# Autodesk Inventor assembly: Assembly_MicroscopeInABox_v0
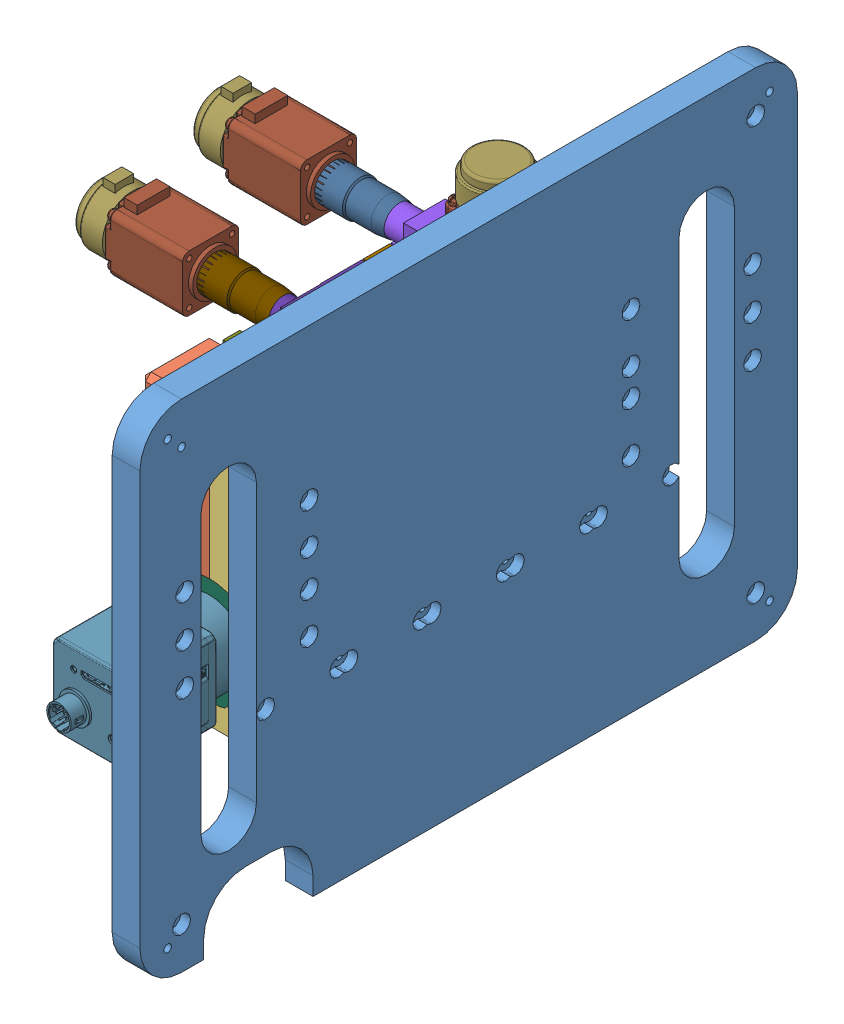
[picture p0: shaded view drawn from the shape stored in the file]
Saved by Autodesk Inventor 2024.1 (Build 281209000, 209)
## iProperties
Created: 2024-08-15
Part Number: Assembly_MicroscopeInABox_v0
Document SubType Name: Assembly
Designer: diederichbenedict
Author: diederichbenedict
## Documents named in this file (9)
- C:\Users\diederichbenedict\Dropbox\Dokumente\Promotion\PROJECTS\openUC2_SOOP\INVENTOR\Workspace\Assembly_MicroscopeInABox_v0.iam
- C:\Users\diederichbenedict\Dropbox\Dokumente\Promotion\PROJECTS\openUC2_SOOP\INVENTOR\Workspace\00_HIKCamera_MV-CE060-10UMUC\00_HIKCamera_MV-CE060-10UMUC.ipt
- C:\Users\diederichbenedict\Dropbox\Dokumente\Promotion\PROJECTS\openUC2_SOOP\INVENTOR\Workspace\00_10x_Objective_ViewSolutions_bm05073332.ipt
- C:\Users\diederichbenedict\Dropbox\Dokumente\Promotion\PROJECTS\openUC2_SOOP\INVENTOR\Workspace\00_Berrybase_CCTVLens_50mm.ipt
- C:\Users\diederichbenedict\Dropbox\Dokumente\Promotion\PROJECTS\openUC2_SOOP\INVENTOR\Workspace\Assembly_XYZ_Stage_Micrometer_ontop_lightsheet.iam
- C:\Users\diederichbenedict\Dropbox\Dokumente\Promotion\PROJECTS\openUC2_SOOP\INVENTOR\Workspace\MIAB_Case_v0.ipt
- C:\Users\diederichbenedict\Dropbox\Dokumente\Promotion\PROJECTS\openUC2_SOOP\INVENTOR\Workspace\MIAB_Case_Opticscube_RMS_1.ipt
- C:\Users\diederichbenedict\Dropbox\Dokumente\Promotion\PROJECTS\openUC2_SOOP\INVENTOR\Workspace\MIAB_Case_v0_MIR.ipt
- C:\Users\diederichbenedict\Dropbox\Dokumente\Promotion\PROJECTS\openUC2_SOOP\INVENTOR\Workspace\60_Planktoscope_MicroscopeHolderXYZ_Bottom_v0.ipt
## Components (8 placed, 8 different names)
1. 00_HIKCamera_MV-CE060-10UMUC:1 — Einfügen:2, Winkel:1
2. 00_10x_Objective_ViewSolutions_bm05073332:1 — Passend:1, Fluchtend:1, Einfügen:1, Passend:2
3. 00_Berrybase_CCTVLens_50mm:1 — Einfügen:1, Einfügen:2, Passend:3
4. Assembly_XYZ_Stage_Micrometer_ontop_lightsheet:1 [sub-assembly] — Passend:2, Winkel:2, Passend:3
5. MIAB_Case_v0:1 — Fluchtend:2, Fluchtend:3, Fluchtend:4, Fluchtend:5, Passend:6, Fluchtend:6, Fluchtend:7
6. MIAB_Case_Opticscube_RMS_1:1 — Fluchtend:4, Fluchtend:5
7. MIAB_Case_v0_MIR:1 — Passend:4, Passend:5
8. 60_Planktoscope_MicroscopeHolderXYZ_Bottom_v0:1 — Passend:6, Fluchtend:6, Fluchtend:7
## Relationships (17: Flush 7, Mate 6, Insert 2, Angle 2)
- Passend:1 [Mate]: 00_10x_Objective_ViewSolutions_bm05073332:1
- Fluchtend:1 [Flush]: 00_10x_Objective_ViewSolutions_bm05073332:1
- Einfügen:1 [Insert] (25 mm): 00_10x_Objective_ViewSolutions_bm05073332:1 ↔ 00_Berrybase_CCTVLens_50mm:1
- Einfügen:2 [Insert]: 00_HIKCamera_MV-CE060-10UMUC:1 ↔ 00_Berrybase_CCTVLens_50mm:1
- Winkel:1 [Angle] (0 deg): 00_HIKCamera_MV-CE060-10UMUC:1
- Passend:2 [Mate]: 00_10x_Objective_ViewSolutions_bm05073332:1 ↔ Assembly_XYZ_Stage_Micrometer_ontop_lightsheet:1
- Winkel:2 [Angle] (0 deg): Assembly_XYZ_Stage_Micrometer_ontop_lightsheet:1
- Passend:3 [Mate] (25 mm): 00_Berrybase_CCTVLens_50mm:1 ↔ Assembly_XYZ_Stage_Micrometer_ontop_lightsheet:1
- Fluchtend:2 [Flush]: MIAB_Case_v0:1
- Fluchtend:3 [Flush]: MIAB_Case_v0:1
- Fluchtend:4 [Flush]: MIAB_Case_v0:1 ↔ MIAB_Case_Opticscube_RMS_1:1
- Fluchtend:5 [Flush]: MIAB_Case_v0:1 ↔ MIAB_Case_Opticscube_RMS_1:1
- Passend:4 [Mate]: MIAB_Case_v0_MIR:1
- Passend:5 [Mate]: MIAB_Case_v0_MIR:1
- Passend:6 [Mate] (20 mm): MIAB_Case_v0:1 ↔ 60_Planktoscope_MicroscopeHolderXYZ_Bottom_v0:1
- Fluchtend:6 [Flush] (-15 mm): MIAB_Case_v0:1 ↔ 60_Planktoscope_MicroscopeHolderXYZ_Bottom_v0:1
- Fluchtend:7 [Flush] (80 mm): MIAB_Case_v0:1 ↔ 60_Planktoscope_MicroscopeHolderXYZ_Bottom_v0:1
